# Autodesk Inventor assembly: Full arm
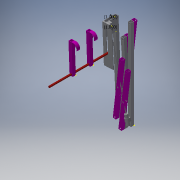
[picture p0: Inventor's stored thumbnail of the model, 180x180]
Saved by Autodesk Inventor 2016 (Build 200138000, 138)
## iProperties
Created: 2016-02-17
Part Number: Full arm
Document SubType Name: Weldment
Designer: Admin
Weld Material: Welded Aluminum-6061
Author: Admin
## Documents named in this file (14)
- C:\Users\Admin\Desktop\robotwithskidplatefeb05\1510-stronghold-CAD-master\arm\Full arm.iam
- C:\Users\Admin\Desktop\robotwithskidplatefeb05\1510-stronghold-CAD-master\arm\AP 1.ipt
- C:\Users\Admin\Desktop\robotwithskidplatefeb05\1510-stronghold-CAD-master\arm\AP 2.ipt
- C:\Users\Admin\Desktop\robotwithskidplatefeb05\1510-stronghold-CAD-master\arm\AP 3.ipt
- C:\Users\Admin\Desktop\robotwithskidplatefeb05\1510-stronghold-CAD-master\arm\AP 4.ipt
- C:\Users\Admin\Desktop\robotwithskidplatefeb05\1510-stronghold-CAD-master\arm\AP 5.ipt
- C:\Users\Admin\Desktop\robotwithskidplatefeb05\1510-stronghold-CAD-master\arm\AP 6.ipt
- C:\Users\Admin\Desktop\robotwithskidplatefeb05\1510-stronghold-CAD-master\arm\Plate.ipt
- C:\Users\Admin\Desktop\robotwithskidplatefeb05\1510-stronghold-CAD-master\arm\Plate add on.ipt
- C:\Users\Admin\Desktop\robotwithskidplatefeb05\1510-stronghold-CAD-master\arm\Hex Shaft.ipt
- C:\Users\Admin\Desktop\robotwithskidplatefeb05\1510-stronghold-CAD-master\arm\claw.ipt
- C:\Users\Admin\Desktop\robotwithskidplatefeb05\1510-stronghold-CAD-master\arm\motor and screw.ipt
- C:\Users\Admin\Desktop\robotwithskidplatefeb05\1510-stronghold-CAD-master\arm\motor spinner.ipt
- C:\Users\Admin\Desktop\robotwithskidplatefeb05\1510-stronghold-CAD-master\arm\Spinner.ipt
## Components (16 placed, 13 different names)
1. AP 1:1 — Flush:1, Flush:2, Mate:2, Mate:19, Flush:3, Mate:27, Mate:29, Mate:34, Mate:41, Mate:56, Mate:64
2. AP 2:1 — Flush:3, Mate:25, Mate:28, Mate:32
3. AP 3:1 — Flush:2, Mate:26, Mate:31, Mate:36, Flush:4, Flush:5
4. AP 4:1 — Flush:1, Mate:22, Mate:33, Mate:35
5. AP 5:1 — Mate:2, Mate:19, Mate:22, Mate:32
6. AP 5:2 — Mate:25, Mate:26, Mate:27
7. AP 5:3 — Mate:28, Mate:29, Mate:31, Mate:33
8. AP 6:1 — Mate:34, Mate:35, Mate:41
9. Plate:1 — Mate:36, Flush:4, Flush:5, Flush:8, Mate:37, Flush:9
10. Plate add on:1 — Flush:8, Mate:37, Flush:9, Mate:38, Mate:39, Flush:10, Mate:46, Mate:68
11. Hex Shaft:1 — Mate:38, Mate:39, Flush:10, Mate:57, Mate:60, Mate:61, Mate:67, Mate:68
12. claw:1 — Mate:49, Mate:60, Mate:61
13. claw:2 — Mate:46, Mate:49, Mate:57, Mate:67
14. motor and screw:1 — Mate:65, Flush:11
15. motor spinner:1 — Mate:63, Mate:64, Mate:65, Flush:11, Mate:66
16. Spinner:1 — Mate:56, Mate:63, Mate:66
## Relationships (39: Mate 30, Flush 9)
- Flush:1: AP 1:1 ↔ AP 4:1
- Flush:2: AP 1:1 ↔ AP 3:1
- Mate:2: AP 1:1 ↔ AP 5:1
- Mate:19: AP 1:1 ↔ AP 5:1
- Flush:3: AP 1:1 ↔ AP 2:1
- Mate:22: AP 4:1 ↔ AP 5:1
- Mate:25: AP 2:1 ↔ AP 5:2
- Mate:26: AP 3:1 ↔ AP 5:2
- Mate:27: AP 1:1 ↔ AP 5:2
- Mate:28: AP 2:1 ↔ AP 5:3
- Mate:29: AP 1:1 ↔ AP 5:3
- Mate:31: AP 3:1 ↔ AP 5:3
- Mate:32: AP 2:1 ↔ AP 5:1
- Mate:33: AP 4:1 ↔ AP 5:3
- Mate:34: AP 1:1 ↔ AP 6:1
- Mate:35: AP 4:1 ↔ AP 6:1
- Mate:36: AP 3:1 ↔ Plate:1
- Flush:4: AP 3:1 ↔ Plate:1
- Flush:5: AP 3:1 ↔ Plate:1
- Flush:8: Plate:1 ↔ Plate add on:1
- Mate:37: Plate:1 ↔ Plate add on:1
- Flush:9: Plate:1 ↔ Plate add on:1
- Mate:38: Plate add on:1 ↔ Hex Shaft:1
- Mate:39: Plate add on:1 ↔ Hex Shaft:1
- Flush:10 (-25.4 mm): Plate add on:1 ↔ Hex Shaft:1
- Mate:41: AP 1:1 ↔ AP 6:1
- Mate:46 (127 mm): Plate add on:1 ↔ claw:2
- Mate:49 (118.618 mm): claw:1 ↔ claw:2
- Mate:56: AP 1:1 ↔ Spinner:1
- Mate:57: Hex Shaft:1 ↔ claw:2
- Mate:60: Hex Shaft:1 ↔ claw:1
- Mate:61: Hex Shaft:1 ↔ claw:1
- Mate:63: motor spinner:1 ↔ Spinner:1
- Mate:64: AP 1:1 ↔ motor spinner:1
- Mate:65: motor and screw:1 ↔ motor spinner:1
- Flush:11 (-25.4 mm): motor and screw:1 ↔ motor spinner:1
- Mate:66: motor spinner:1 ↔ Spinner:1
- Mate:67: Hex Shaft:1 ↔ claw:2
- Mate:68: Plate add on:1 ↔ Hex Shaft:1
